# Autodesk Inventor assembly: Front Bumper1
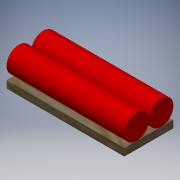
[picture p0: Inventor's stored thumbnail of the model, 180x180]
Saved by Autodesk Inventor 2018 (Build 220112000, 112)
## iProperties
Created: 2018-01-17
Part Number: Front Bumper1
Document SubType Name: Assembly
Designer: Apple
Author: Apple
## Documents named in this file (4)
- C:\Users\Apple\Documents\Inventor\2018 PowerUp\Bumper\Front Bumper1.iam
- C:\Users\Apple\Documents\Inventor\2018 PowerUp\Bumper\Front Board.ipt
- C:\Users\Apple\Documents\Inventor\2018 PowerUp\Bumper\Front Noodle 1.ipt
- C:\Users\Apple\Documents\Inventor\2018 PowerUp\Bumper\Front Noodle 2.ipt
## Components (3 placed, 3 different names)
1. Front Board:1 — Flush:1, Flush:2
2. Front Noodle 1:1 — Flush:1
3. Front Noodle 2:1 — Flush:2
## Relationships (2: Flush 2)
- Flush:1: Front Board:1 ↔ Front Noodle 1:1
- Flush:2: Front Board:1 ↔ Front Noodle 2:1
